# Autodesk Inventor assembly: 211-07
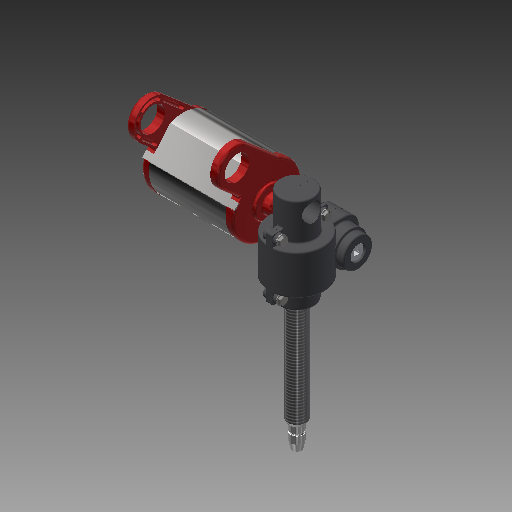
[picture p0: Inventor's stored thumbnail of the model, 512x512]
Saved by Autodesk Inventor 2019 (Build 230136000, 136)
## iProperties
Company: Autodesk Inc.
Created: 2008-01-21
Part Number: 211-07
Document SubType Name: Assembly
Designer: Autodesk Inc.
Description: WORM DRIVE ASSEMBLY
Mass: 248.247 g
Surface Area: 732.521 cm^2
Volume: 92.845 cm^3
Density: 2.67378 g/cm^3
Author: Inventor
## Documents named in this file (4)
- C:\TEMP\Car Seat\Workspace\Rear Worm Drive Assembly.iam
- C:\TEMP\Car Seat\Workspace\Rear Worm Drive.iam
- C:\TEMP\Car Seat\Workspace\Rear Ball Screw Shaft Assembly.iam
- C:\TEMP\Car Seat\Workspace\Rear Worm Motor Shaft.iam
## Components (3 placed, 3 different names)
1. Rear Worm Drive:1 [sub-assembly] — Insert:1, Insert:2
2. Rear Worm Drive Shaft:1 [sub-assembly] — Insert:1
3. Rear Worm Motor Shaft:1 [sub-assembly] — Insert:2
## Relationships (2: Insert 2)
- Insert:1: Rear Worm Drive:1 ↔ Rear Worm Drive Shaft:1
- Insert:2: Rear Worm Drive:1 ↔ Rear Worm Motor Shaft:1
